# Autodesk Inventor assembly: shooter
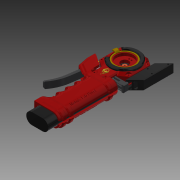
[picture p0: Inventor's stored thumbnail of the model, 180x180]
Saved by Autodesk Inventor 2018 (Build 220112000, 112)
## iProperties
Created: 2019-02-20
Part Number: shooter
Material: 一般
Document SubType Name: Assembly
Designer: ku_sk
Author: ku_sk
## Documents named in this file (14)
- E:\windows\InventorProjects\BayBlade_Launcher\Launcher.iam
- E:\windows\InventorProjects\BayBlade_Launcher\parts\bay conect.ipt
- E:\windows\InventorProjects\BayBlade_Launcher\parts\gear.ipt
- E:\windows\InventorProjects\BayBlade_Launcher\parts\undercover.ipt
- E:\windows\InventorProjects\BayBlade_Launcher\parts\bearing.ipt
- E:\windows\InventorProjects\BayBlade_Launcher\parts\battery.ipt
- E:\windows\InventorProjects\BayBlade_Launcher\parts\brake.ipt
- E:\windows\InventorProjects\BayBlade_Launcher\parts\bar.ipt
- E:\windows\InventorProjects\BayBlade_Launcher\parts\switch.ipt
- E:\windows\InventorProjects\BayBlade_Launcher\parts\joint.ipt
- E:\windows\InventorProjects\BayBlade_Launcher\parts\circuitcover.ipt
- E:\windows\InventorProjects\BayBlade_Launcher\parts\circuitcover1.ipt
- E:\windows\InventorProjects\BayBlade_Launcher\parts\pushbar.ipt
- E:\windows\InventorProjects\BayBlade_Launcher\parts\toptest.iam
## Components (16 placed, 13 different names)
1. bay conect:1 — メイト:1, フラッシュ:1, メイト:2, メイト:3, メイト:7, メイト:8, メイト:9, メイト:13
2. gear:1 — メイト:2, メイト:3
3. undercover:1 — フラッシュ:3, メイト:7, フラッシュ:4, メイト:12, メイト:14, 正接:1, メイト:22, メイト:28, 角度:1, メイト:29, メイト:30, メイト:32, メイト:33, メイト:34, フラッシュ:10, メイト:40, フラッシュ:11
4. bearing:1 — メイト:8, メイト:9, フラッシュ:4
5. battery:1 — メイト:28, 角度:1, メイト:29, メイト:33
6. bar:1 — メイト:13, メイト:14, メイト:15, メイト:24, メイト:41
7. joint:1 — メイト:24, メイト:25
8. circuitcover:1 — メイト:30, メイト:32, メイト:34, メイト:35, フラッシュ:8, フラッシュ:9
9. circuitcover1:1 — メイト:35, フラッシュ:8, フラッシュ:9
10. switch:1 — メイト:22, メイト:25, フラッシュ:10, メイト:37, メイト:38, メイト:39
11. pushbar:1 — メイト:37, メイト:38, メイト:39
12. toptest:1 [sub-assembly] — メイト:40, メイト:41, フラッシュ:11
13. brake:1 — メイト:12, メイト:15, 正接:1
14. brake:2
15. brake:3
16. brake:4
## Component patterns: (4 elements, first: brake:1)
## Relationships (34: Mate 25, Flush 7, Tangent 1, Angle 1)
- メイト:1 [Mate]: bay conect:1
- フラッシュ:1 [Flush]: bay conect:1
- メイト:2 [Mate]: bay conect:1 ↔ gear:1
- メイト:3 [Mate]: bay conect:1 ↔ gear:1
- フラッシュ:3 [Flush]: undercover:1
- メイト:7 [Mate]: bay conect:1 ↔ undercover:1
- メイト:8 [Mate]: bay conect:1 ↔ bearing:1
- メイト:9 [Mate]: bay conect:1 ↔ bearing:1
- フラッシュ:4 [Flush]: undercover:1 ↔ bearing:1
- メイト:12 [Mate] (1.75 mm): undercover:1 ↔ brake:1
- メイト:13 [Mate]: bay conect:1 ↔ bar:1
- メイト:14 [Mate]: undercover:1 ↔ bar:1
- メイト:15 [Mate]: bar:1 ↔ brake:1
- 正接:1 [Tangent]: undercover:1 ↔ brake:1
- メイト:22 [Mate] (0.5 mm): undercover:1 ↔ switch:1
- メイト:24 [Mate]: bar:1 ↔ joint:1
- メイト:25 [Mate]: joint:1 ↔ switch:1
- メイト:28 [Mate]: undercover:1 ↔ battery:1
- 角度:1 [Angle] (0 deg): undercover:1 ↔ battery:1
- メイト:29 [Mate] (-0.5 mm): undercover:1 ↔ battery:1
- メイト:30 [Mate]: undercover:1 ↔ circuitcover:1
- メイト:32 [Mate]: undercover:1 ↔ circuitcover:1
- メイト:33 [Mate] (0.5 mm): undercover:1 ↔ battery:1
- メイト:34 [Mate]: undercover:1 ↔ circuitcover:1
- メイト:35 [Mate]: circuitcover:1 ↔ circuitcover1:1
- フラッシュ:8 [Flush]: circuitcover:1 ↔ circuitcover1:1
- フラッシュ:9 [Flush]: circuitcover:1 ↔ circuitcover1:1
- フラッシュ:10 [Flush] (4.5 mm): undercover:1 ↔ switch:1
- メイト:37 [Mate]: switch:1 ↔ pushbar:1
- メイト:38 [Mate]: switch:1 ↔ pushbar:1
- メイト:39 [Mate]: switch:1 ↔ pushbar:1
- メイト:40 [Mate]: undercover:1 ↔ toptest:1
- メイト:41 [Mate]: bar:1 ↔ toptest:1
- フラッシュ:11 [Flush]: undercover:1 ↔ toptest:1
